# Autodesk Inventor assembly: main
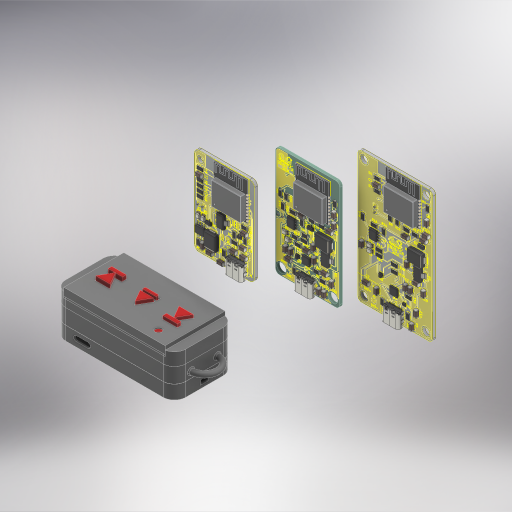
[picture p0: Inventor's stored thumbnail of the model, 512x512]
Saved by Autodesk Inventor 2024.4 (Build 284460000, 460)
## iProperties
Created: 2025-07-27
Part Number: main
Document SubType Name: Assembly
Designer: User
Author: User
## Documents named in this file (14)
- C:\Users\Duszy\Desktop\Projekty\Clickfy\Clickfy_V1\main.iam
- C:\Users\Duszy\Downloads\esp32-wroom-32-3.snapshot.8\esp32_30pin\esp32_30pin\esp32_30pin.iam
- C:\Users\Duszy\Downloads\Micro_Button_6x6\Micro_Button_6x6\Micro_Button_6x6.ipt
- C:\Users\Duszy\Downloads\tp4056-charging-module-type-c-1.snapshot.1\TP4056_Charging_Module_Type_C\TP4056_Charging_Module_Type_C\TP4056_Charging_Module_Type_C.ipt
- C:\Users\Duszy\Desktop\Projekty\Clickfy\Clickfy_V1\bateria_prop.ipt
- C:\Users\Duszy\Desktop\Projekty\Clickfy\Clickfy_V1\rama.ipt
- C:\Users\Duszy\Desktop\Projekty\Clickfy\Clickfy_V1\flor.ipt
- C:\Users\Duszy\Desktop\Projekty\Clickfy\Clickfy_V1\button_bottom.ipt
- C:\Users\Duszy\Desktop\Projekty\Clickfy\Clickfy_V1\button_top.ipt
- C:\Users\Duszy\Desktop\Projekty\Clickfy\Clickfy_V1\guzik.ipt
- C:\Users\Duszy\Desktop\Projekty\Clickfy\Clickfy_V1\guzik_szablon.ipt
- C:\Users\Duszy\Desktop\Projekty\Clickfy\Clickfy_V2\Clickfy_v2\Clickfy.kicad_v1_pcb\Clickfy.kicad_v1_pcb.ipt
- C:\Users\Duszy\Desktop\Projekty\Clickfy\Clickfy_V2\Clickfy_v2\Clickfy_v3\Clickfy_v3.ipt
- C:\Users\Duszy\Desktop\Projekty\Clickfy\Clickfy_V2\Clickfy_v2\Clickfy_v2\Clickfy_v2.ipt
## Components (16 placed, 13 different names)
1. esp32_30pin:1 [sub-assembly] — Obrotowe:1
2. Micro_Button_6x6:1 — Sztywne:3, Obrotowe:4
3. Micro_Button_6x6:2 — Sztywne:4
4. Micro_Button_6x6:3 — Sztywne:2, Obrotowe:3
5. TP4056_Charging_Module_Type_C:1 — Sztywne:1
6. bateria_prop:1 — przesuwne:1
7. rama:1 — przesuwne:1, Sztywne:1, Obrotowe:2, Sztywne:5
8. flor:1 — Obrotowe:1, Obrotowe:2
9. button_bottom:1 — Sztywne:2, Sztywne:3, Sztywne:4, Sztywne:5
10. button_top:1 — Obrotowe:5, Sztywne:6
11. guzik:1 — Obrotowe:3, Obrotowe:5
12. guzik_szablon:1 — Obrotowe:4
13. guzik:2 — Sztywne:6
14. Clickfy.kicad_v1_pcb:1
15. Clickfy_v3:1
16. Clickfy_v2:1
## Relationships (12: WeldJoint 6, RevoluteJoint 5, TranslationJoint 1)
- przesuwne:1 [TranslationJoint] (0.3 mm): bateria_prop:1 ↔ rama:1
- Sztywne:1 [WeldJoint] (0.15 mm): TP4056_Charging_Module_Type_C:1 ↔ rama:1
- Obrotowe:1 [RevoluteJoint] (0.1 mm): esp32_30pin:1 ↔ flor:1
- Obrotowe:2 [RevoluteJoint] (-7.35 mm): rama:1 ↔ flor:1
- Sztywne:2 [WeldJoint]: Micro_Button_6x6:3 ↔ button_bottom:1
- Sztywne:3 [WeldJoint]: Micro_Button_6x6:1 ↔ button_bottom:1
- Sztywne:4 [WeldJoint]: Micro_Button_6x6:2 ↔ button_bottom:1
- Sztywne:5 [WeldJoint] (-15.45 mm): rama:1 ↔ button_bottom:1
- Obrotowe:3 [RevoluteJoint]: Micro_Button_6x6:3 ↔ guzik:1
- Obrotowe:4 [RevoluteJoint]: Micro_Button_6x6:1 ↔ guzik_szablon:1
- Obrotowe:5 [RevoluteJoint] (-2 mm): button_top:1 ↔ guzik:1
- Sztywne:6 [WeldJoint] (2 mm): button_top:1 ↔ guzik:2
